# Autodesk Inventor assembly: Chasis
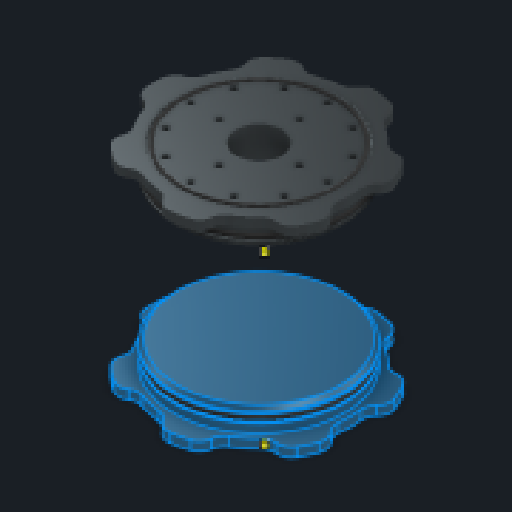
[picture p0: Inventor's stored thumbnail of the model, 512x512]
Saved by Autodesk Inventor 2025.3 (Build 293356030, 356C)
## iProperties
Created: 2024-12-25
Part Number: Chasis
Document SubType Name: Assembly
Designer: Usuario
Author: Usuario
## Documents named in this file (6)
- C:\Users\santa\OneDrive - Universidad de los Andes\Robocol\Flotador\V3\Chasis.iam
- C:\Users\santa\OneDrive - Universidad de los Andes\Robocol\Flotador\V3\Chasis\Tapa_Inferior.ipt
- C:\Users\santa\OneDrive - Universidad de los Andes\Robocol\Flotador\V3\Chasis\Tapa_Superior.ipt
- C:\Users\santa\OneDrive - Universidad de los Andes\Robocol\Flotador\V3\Chasis\Tuberia.ipt
- C:\Users\santa\OneDrive - Universidad de los Andes\Robocol\Flotador\V3\O'Ring\1.78.ipt
- C:\Users\santa\OneDrive - Universidad de los Andes\Robocol\Flotador\V3\O'Ring\2.62.ipt
## Components (6 placed, 5 different names)
1. Tuberia:1 — Rígido:1, Rígido:2, Nivelación:1, Nivelación:2, Nivelación:3
2. Tapa_Inferior:1 — Rígido:2, Rígido:5
3. Tapa_Superior:1 — Rígido:1, Rígido:3, Rígido:4
4. 1.78:1 — Rígido:4
5. 2.62:1 — Rígido:3
6. 2.62:2 — Rígido:5
## Relationships (8: WeldJoint 5, Flush 3)
- Rígido:1 [WeldJoint]: Tuberia:1 ↔ Tapa_Superior:1
- Rígido:2 [WeldJoint]: Tuberia:1 ↔ Tapa_Inferior:1
- Nivelación:1 [Flush]: Tuberia:1
- Nivelación:2 [Flush]: Tuberia:1
- Nivelación:3 [Flush]: Tuberia:1
- Rígido:3 [WeldJoint]: Tapa_Superior:1 ↔ 2.62:1
- Rígido:4 [WeldJoint] (0.89 mm): Tapa_Superior:1 ↔ 1.78:1
- Rígido:5 [WeldJoint]: Tapa_Inferior:1 ↔ 2.62:2
